# Autodesk Inventor assembly: Montagem Motor
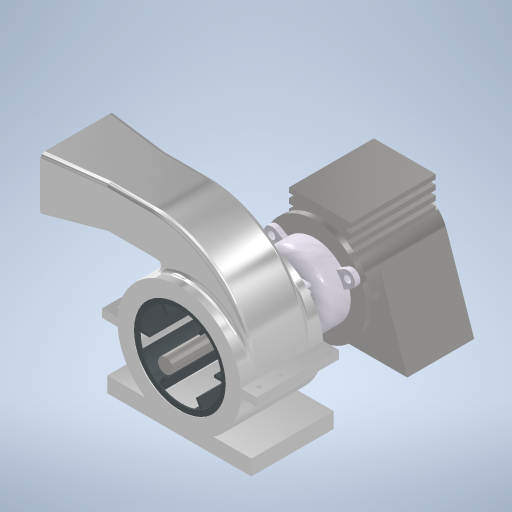
[picture p0: Inventor's stored thumbnail of the model, 512x512]
Saved by Autodesk Inventor 2023.2 (Build 272271000, 271)
## iProperties
Created: 2022-12-18
Part Number: Montagem Motor
Document SubType Name: Assembly
Designer: coqui
Author: coqui
## Documents named in this file (7)
- D:\Felipe Coquito\OneDrive\Documents\Inventor\Inventor - curso\Montagem\Montagem Motor.iam
- D:\Felipe Coquito\OneDrive\Documents\Inventor\Inventor - curso\Motor Industrial\Carcaça Inferior do Motor Industiral.ipt
- D:\Felipe Coquito\OneDrive\Documents\Inventor\Inventor - curso\Motor Industrial\Cilindro do Motor Industrial.ipt
- D:\Felipe Coquito\OneDrive\Documents\Inventor\Inventor - curso\Motor Industrial\Carcaça Superior do Motor Industrial.ipt
- D:\Felipe Coquito\OneDrive\Documents\Inventor\Inventor - curso\Motor Industrial\Disco do Motor Industrial.ipt
- D:\Felipe Coquito\OneDrive\Documents\Inventor\Inventor - curso\Motor Industrial\Base do Motor Industrial.ipt
- D:\Felipe Coquito\OneDrive\Documents\Inventor\Inventor - curso\Motor Industrial\Eixo do Motor Industrial.ipt
## Components (6 placed, 6 different names)
1. Carcaça Inferior do Motor Industiral:1 — Mate:1, Mate:2, Mate:3, Mate:9
2. Cilindro do Motor Industrial:1 — Mate:1, Mate:2, Mate:4, Mate:5
3. Carcaça Superior do Motor Industrial:1 — Mate:3, Mate:9
4. Disco do Motor Industrial:1 — Mate:4, Mate:5, Mate:6, Mate:7, Mate:8
5. Base do Motor Industrial:1 — Mate:6, Mate:7, Mate:8, Mate:10, Mate:11
6. Eixo do Motor Industrial:1 — Mate:10, Mate:11
## Relationships (11: Mate 11)
- Mate:1: Carcaça Inferior do Motor Industiral:1 ↔ Cilindro do Motor Industrial:1
- Mate:2: Carcaça Inferior do Motor Industiral:1 ↔ Cilindro do Motor Industrial:1
- Mate:3: Carcaça Inferior do Motor Industiral:1 ↔ Carcaça Superior do Motor Industrial:1
- Mate:4: Cilindro do Motor Industrial:1 ↔ Disco do Motor Industrial:1
- Mate:5: Cilindro do Motor Industrial:1 ↔ Disco do Motor Industrial:1
- Mate:6: Disco do Motor Industrial:1 ↔ Base do Motor Industrial:1
- Mate:7: Disco do Motor Industrial:1 ↔ Base do Motor Industrial:1
- Mate:8: Disco do Motor Industrial:1 ↔ Base do Motor Industrial:1
- Mate:9: Carcaça Inferior do Motor Industiral:1 ↔ Carcaça Superior do Motor Industrial:1
- Mate:10: Base do Motor Industrial:1 ↔ Eixo do Motor Industrial:1
- Mate:11: Base do Motor Industrial:1 ↔ Eixo do Motor Industrial:1
